# Autodesk Inventor assembly: Left Hook Whole Assembly_v2
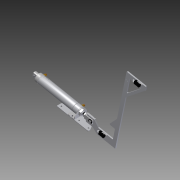
[picture p0: Inventor's stored thumbnail of the model, 180x180]
Saved by Autodesk Inventor 2014 SP1 (Build 180222100, 222)
## iProperties
Created: 2013-03-16
Part Number: Left Hook Whole Assembly_v2
Document SubType Name: Assembly
Designer: Arpan
Mass: 1491.03 g
Surface Area: 1681.51 cm^2
Volume: 296.561 cm^3
Density: 5.02773 g/cm^3
Author: Arpan
## Documents named in this file (4)
- C:\Users\Moses\Documents\Inventor\Sally Rebuild\Rebuild Sally\Left Hook Whole Assembly_v2.iam
- C:\Users\Moses\Documents\Inventor\Sally Rebuild\Rebuild Sally\Left Hook Encoder Assembly.iam
- C:\Users\Moses\Documents\Inventor\Sally Rebuild\Rebuild Sally\Ninja left cylinder support bracket.ipt
- C:\Users\Moses\Documents\Inventor\Sally Rebuild\Rebuild Sally\Piston Bracket Assembly - L.iam
## Components (3 placed, 3 different names)
1. Left Hook Encoder Assembly:1 [sub-assembly] — Mate:7, Mate:8, Mate:9
2. Piston Bracket Assembly - L:1 [sub-assembly] — Mate:7, Mate:8, Mate:9, Mate:10, Mate:11, Mate:12
3. Ninja left cylinder support bracket:1 — Mate:10, Mate:11, Mate:12
## Relationships (6: Mate 6)
- Mate:7: Left Hook Encoder Assembly:1 ↔ Piston Bracket Assembly - L:1
- Mate:8: Left Hook Encoder Assembly:1 ↔ Piston Bracket Assembly - L:1
- Mate:9: Left Hook Encoder Assembly:1 ↔ Piston Bracket Assembly - L:1
- Mate:10: Piston Bracket Assembly - L:1 ↔ Ninja left cylinder support bracket:1
- Mate:11: Piston Bracket Assembly - L:1 ↔ Ninja left cylinder support bracket:1
- Mate:12: Piston Bracket Assembly - L:1 ↔ Ninja left cylinder support bracket:1
